# Autodesk Inventor assembly: House_Assembly
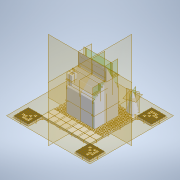
[picture p0: Inventor's stored thumbnail of the model, 180x180]
Saved by Autodesk Inventor 2022.4 (Build 264492010, 492A)
## iProperties
Created: 2025-02-20
Part Number: House_Assembly
Document SubType Name: Assembly
Designer: jan-m
Author: jan-m
## Documents named in this file (21)
- C:\School\Masterproef\3D Modellen\House_Assembly.iam
- C:\School\Masterproef\3D Modellen\Tile.ipt
- C:\School\Masterproef\3D Modellen\Tile_Connector.ipt
- C:\School\Masterproef\3D Modellen\Wall.ipt
- C:\School\Masterproef\3D Modellen\Roof_Wall_Small_Left.ipt
- C:\School\Masterproef\3D Modellen\Roof_Wall_Small_Right.ipt
- C:\School\Masterproef\3D Modellen\Roof_Wall_Large_Left.ipt
- C:\School\Masterproef\3D Modellen\Roof_Wall_Large_Right.ipt
- C:\School\Masterproef\3D Modellen\Roof_Small.ipt
- C:\School\Masterproef\3D Modellen\Roof_Large.ipt
- C:\School\Masterproef\3D Modellen\Hanging_Wall.ipt
- C:\School\Masterproef\3D Modellen\1x1_Piece.ipt
- C:\School\Masterproef\3D Modellen\Marker_Tile.ipt
- C:\School\Masterproef\3D Modellen\Tile_Cover.ipt
- C:\School\Masterproef\3D Modellen\Tree_Leaves.ipt
- C:\School\Masterproef\3D Modellen\Tree_Trunk.ipt
- C:\School\Masterproef\3D Modellen\Chimney.ipt
- C:\School\Masterproef\3D Modellen\Pin.ipt
- C:\School\Masterproef\3D Modellen\Rail_Clip_Left.ipt
- C:\School\Masterproef\3D Modellen\Rail_Clip_Right.ipt
- C:\School\Masterproef\3D Modellen\Roof_Pin_Clip.ipt
## Components (403 placed, 20 different names)
1. Wall:1 — Mate:10, Mate:11, Mate:12, Mate:40, Mate:46, Mate:59
2. Wall:2 — Mate:13, Mate:14, Mate:15, Mate:27, Mate:28, Mate:30, Mate:31, Mate:60, Mate:64, Mate:72
3. Wall:3 — Mate:19, Mate:20, Mate:21, Mate:37, Mate:42, Mate:58
4. Wall:4 — Mate:16, Mate:17, Mate:18, Mate:23, Mate:25, Mate:33, Mate:34, Mate:63, Mate:65
5. Roof_Wall_Small_Left:2 — Mate:23, Mate:25, Mate:65, Mate:80, Mate:81, Flush:6, Mate:102, Flush:12, Angle:1
6. Roof_Wall_Small_Right:2 — Mate:27, Mate:28, Mate:64, Mate:72, Mate:101, Mate:103, Flush:13, Angle:2
7. Roof_Wall_Large_Left:1 — Mate:30, Mate:31, Mate:60, Mate:106, Flush:16, Angle:5, Mate:107, Flush:17, Angle:6
8. Roof_Wall_Large_Right:1 — Mate:33, Mate:34, Mate:63, Mate:98, Mate:104, Flush:14, Angle:3, Mate:105, Flush:15, Angle:4
9. Roof_Small:1 — Mate:37, Mate:42, Mate:58, Mate:96, Mate:97, Mate:99, Mate:100
10. Roof_Large:1 — Mate:40, Mate:43, Mate:44, Mate:46, Mate:59, Flush:7
11. Hanging_Wall:1 — Mate:43, Mate:44, Flush:7
12. Tree_Leaves:1 — Mate:73, Mate:74
13. Tree_Trunk:1 — Mate:73, Mate:74, Mate:75, Mate:76, Mate:77
14. Chimney:1 — Mate:78, Mate:79, Mate:81, Flush:6
15. Pin:1 — Mate:78, Mate:79, Mate:80
16. Rail_Clip_Left:1 — Mate:96, Mate:97, Mate:98
17. Rail_Clip_Right:1 — Mate:99, Mate:100, Mate:101
18. Roof_Pin_Clip:1 — Mate:105, Flush:15, Angle:4
19. Roof_Pin_Clip:2 — Mate:106, Flush:16, Angle:5
20. Roof_Pin_Clip:3 — Mate:104, Flush:14, Angle:3
21. Roof_Pin_Clip:4 — Mate:102, Flush:12, Angle:1
22. Roof_Pin_Clip:5 — Mate:107, Flush:17, Angle:6
23. Roof_Pin_Clip:6 — Mate:103, Flush:13, Angle:2
24. Tile_Connector:2 — Mate:6, Mate:7
25. Tile:1 — Mate:2, Mate:5, Mate:6, Mate:7, Mate:16, Mate:91, Mate:92
26. Tile_Connector:1 — Mate:2, Mate:5
27. Tile_Connector:3
28. Tile:2 — Mate:10, Mate:12
29. Tile_Connector:4
30. Tile_Connector:5
31. Tile:3 — Mate:11
32. Tile_Connector:6
33. Tile_Connector:7
34. Tile:4 — Mate:13, Mate:75, Mate:76, Mate:77, Mate:94, Mate:95, Flush:11
35. Tile_Connector:8
36. Tile_Connector:9
37. Tile:5
38. Tile_Connector:10
39. Tile_Connector:11
40. Tile:6
41. Tile_Connector:12
42. Tile_Connector:13
43. Tile:7 — Mate:82, Flush:9
44. Tile_Connector:14
45. Tile_Connector:15
46. Tile:8 — Mate:15
47. Tile_Connector:16
48. Tile_Connector:17
49. Tile:9 — Mate:17, Mate:18, Mate:83, Mate:84, Flush:10, Mate:85, Mate:86
50. Tile_Connector:18
51. Tile_Connector:19
52. Tile:10 — Mate:19, Mate:21
53. Tile_Connector:20
54. Tile_Connector:21
55. Tile:11 — Mate:20
56. Tile_Connector:22
57. Tile_Connector:23
58. Tile:12 — Mate:14, Mate:88, Mate:89
59. Tile_Connector:24
60. Tile_Connector:25
61. Tile:13 — Mate:57, Mate:61, Mate:62
62. Tile_Connector:26
63. Tile_Connector:27
64. Tile:14
65. Tile_Connector:28
66. Tile_Connector:29
67. Tile:15
68. Tile_Connector:30
69. Tile_Connector:31
70. Tile:16 — Mate:66, Mate:68, Mate:70
71. Tile_Connector:32
72. Marker_Tile:1 — Mate:53, Mate:54, Flush:5, Mate:67, Mate:69, Mate:71
73. Tile_Connector:33 — Mate:66, Mate:67, Mate:68, Mate:69, Mate:70, Mate:71
74. Marker_Tile:2
75. Tile_Connector:34
76. Marker_Tile:3
77. Tile_Connector:35
78. Marker_Tile:4
79. Tile_Connector:36
80. Tile_Cover:1 — Mate:57, Mate:61, Mate:62
81. Tile_Cover:2
82. Tile_Cover:3
83. Tile_Cover:4
84. 1x1_Piece:147 — Mate:83, Mate:84, Flush:10
85. 1x1_Piece:155
86. 1x1_Piece:156
87. 1x1_Piece:157 — Mate:87
88. 1x1_Piece:158
89. 1x1_Piece:159
90. 1x1_Piece:160
91. 1x1_Piece:161
92. 1x1_Piece:162
93. 1x1_Piece:163
94. 1x1_Piece:164
95. 1x1_Piece:165
96. 1x1_Piece:166
97. 1x1_Piece:167
98. 1x1_Piece:168
99. 1x1_Piece:169
100. 1x1_Piece:170
101. 1x1_Piece:171
102. 1x1_Piece:172
103. 1x1_Piece:173
104. 1x1_Piece:174
105. 1x1_Piece:175
106. 1x1_Piece:176
107. 1x1_Piece:177
108. 1x1_Piece:178
109. 1x1_Piece:179
110. 1x1_Piece:180
111. 1x1_Piece:181
112. 1x1_Piece:182
113. 1x1_Piece:183
114. 1x1_Piece:184
115. 1x1_Piece:185
116. 1x1_Piece:186
117. 1x1_Piece:187
118. 1x1_Piece:188
119. 1x1_Piece:189
120. 1x1_Piece:190
121. 1x1_Piece:191
122. 1x1_Piece:192
123. 1x1_Piece:193
124. 1x1_Piece:194
125. 1x1_Piece:195
126. 1x1_Piece:196
127. 1x1_Piece:197
128. 1x1_Piece:198
129. 1x1_Piece:199
130. 1x1_Piece:200
131. 1x1_Piece:201 — Mate:93
132. 1x1_Piece:202
133. 1x1_Piece:203
134. 1x1_Piece:204
135. 1x1_Piece:205
136. 1x1_Piece:206
137. 1x1_Piece:207
138. 1x1_Piece:208
139. 1x1_Piece:209
140. 1x1_Piece:210
141. 1x1_Piece:211
142. 1x1_Piece:212
143. 1x1_Piece:213
144. 1x1_Piece:146 — Mate:85, Mate:86, Mate:87
145. 1x1_Piece:214
146. 1x1_Piece:215
147. 1x1_Piece:216
148. 1x1_Piece:217
149. 1x1_Piece:218
150. 1x1_Piece:219
151. 1x1_Piece:220
152. 1x1_Piece:221
153. 1x1_Piece:222
154. 1x1_Piece:223
155. 1x1_Piece:224 — Mate:90
156. 1x1_Piece:151 — Mate:88, Mate:89, Mate:90
157. 1x1_Piece:225
158. 1x1_Piece:226
159. 1x1_Piece:227
160. 1x1_Piece:228
161. 1x1_Piece:229
162. 1x1_Piece:230
163. 1x1_Piece:231
164. 1x1_Piece:232
165. 1x1_Piece:233
166. 1x1_Piece:234
167. 1x1_Piece:235
168. 1x1_Piece:236
169. 1x1_Piece:237
170. 1x1_Piece:238
171. 1x1_Piece:239
172. 1x1_Piece:240
173. 1x1_Piece:241
174. 1x1_Piece:242
175. 1x1_Piece:243
176. 1x1_Piece:244
177. 1x1_Piece:245
178. 1x1_Piece:246
179. 1x1_Piece:247
180. 1x1_Piece:248
181. 1x1_Piece:249
182. 1x1_Piece:250
183. 1x1_Piece:251
184. 1x1_Piece:252
185. 1x1_Piece:253
186. 1x1_Piece:254
187. 1x1_Piece:255
188. 1x1_Piece:256
189. 1x1_Piece:257
190. 1x1_Piece:258
191. 1x1_Piece:259
192. 1x1_Piece:260
193. 1x1_Piece:261
194. 1x1_Piece:262
195. 1x1_Piece:263
196. 1x1_Piece:264
197. 1x1_Piece:265
198. 1x1_Piece:266
199. 1x1_Piece:267
200. 1x1_Piece:268
201. 1x1_Piece:269
202. 1x1_Piece:270
203. 1x1_Piece:271
204. 1x1_Piece:272
205. 1x1_Piece:273
206. 1x1_Piece:274
207. 1x1_Piece:275
208. 1x1_Piece:145 — Mate:91, Mate:92, Mate:93
209. 1x1_Piece:276
210. 1x1_Piece:277
211. 1x1_Piece:278
212. 1x1_Piece:279
213. 1x1_Piece:280
214. 1x1_Piece:281
215. 1x1_Piece:282
216. 1x1_Piece:283
217. 1x1_Piece:284
218. 1x1_Piece:285
219. 1x1_Piece:286
220. 1x1_Piece:287
221. 1x1_Piece:288
222. 1x1_Piece:289
223. 1x1_Piece:290
224. 1x1_Piece:291
225. 1x1_Piece:292
226. 1x1_Piece:293
227. 1x1_Piece:294
228. 1x1_Piece:295
229. 1x1_Piece:296
230. 1x1_Piece:297
231. 1x1_Piece:298
232. 1x1_Piece:299
233. 1x1_Piece:300
234. 1x1_Piece:301
235. 1x1_Piece:302
236. 1x1_Piece:303
237. 1x1_Piece:304
238. 1x1_Piece:305
239. 1x1_Piece:306
240. 1x1_Piece:307
241. 1x1_Piece:308
242. 1x1_Piece:309
243. 1x1_Piece:310
244. 1x1_Piece:311
245. 1x1_Piece:312
246. 1x1_Piece:313
247. 1x1_Piece:314
248. 1x1_Piece:315
249. 1x1_Piece:316
250. 1x1_Piece:317
251. 1x1_Piece:318
252. 1x1_Piece:319
253. 1x1_Piece:320
254. 1x1_Piece:321
255. 1x1_Piece:322
256. 1x1_Piece:148 — Mate:94, Mate:95, Flush:11
257. 1x1_Piece:323
258. 1x1_Piece:324
259. 1x1_Piece:325
260. 1x1_Piece:1 — Mate:53, Mate:54, Flush:5, Flush:8
261. 1x1_Piece:2
262. 1x1_Piece:3
263. 1x1_Piece:4
264. 1x1_Piece:5
265. 1x1_Piece:6
266. 1x1_Piece:7
267. 1x1_Piece:8
268. 1x1_Piece:9
269. 1x1_Piece:10
270. 1x1_Piece:11
271. 1x1_Piece:12
272. 1x1_Piece:13
273. 1x1_Piece:14
274. 1x1_Piece:15
275. 1x1_Piece:16
276. 1x1_Piece:17
277. 1x1_Piece:18
278. 1x1_Piece:19
279. 1x1_Piece:20
280. 1x1_Piece:21
281. 1x1_Piece:22
282. 1x1_Piece:23
283. 1x1_Piece:24
284. 1x1_Piece:25
285. 1x1_Piece:26
286. 1x1_Piece:27
287. 1x1_Piece:28
288. 1x1_Piece:29
289. 1x1_Piece:30
290. 1x1_Piece:31
291. 1x1_Piece:32
292. 1x1_Piece:33
293. 1x1_Piece:34
294. 1x1_Piece:35
295. 1x1_Piece:36
296. 1x1_Piece:37
297. 1x1_Piece:38
298. 1x1_Piece:39
299. 1x1_Piece:40
300. 1x1_Piece:41
301. 1x1_Piece:42
302. 1x1_Piece:43
303. 1x1_Piece:44
304. 1x1_Piece:45
305. 1x1_Piece:46
306. 1x1_Piece:47
307. 1x1_Piece:48
308. 1x1_Piece:49
309. 1x1_Piece:50
310. 1x1_Piece:51
311. 1x1_Piece:52
312. 1x1_Piece:53
313. 1x1_Piece:54
314. 1x1_Piece:55
315. 1x1_Piece:56
316. 1x1_Piece:57
317. 1x1_Piece:58
318. 1x1_Piece:59
319. 1x1_Piece:60
320. 1x1_Piece:61
321. 1x1_Piece:62
322. 1x1_Piece:63
323. 1x1_Piece:64
324. 1x1_Piece:65
325. 1x1_Piece:66
326. 1x1_Piece:67
327. 1x1_Piece:68
328. 1x1_Piece:69
329. 1x1_Piece:70
330. 1x1_Piece:71
331. 1x1_Piece:72
332. 1x1_Piece:73
333. 1x1_Piece:74
334. 1x1_Piece:75
335. 1x1_Piece:76
336. 1x1_Piece:77
337. 1x1_Piece:78
338. 1x1_Piece:79
339. 1x1_Piece:80
340. 1x1_Piece:81
341. 1x1_Piece:82
342. 1x1_Piece:83
343. 1x1_Piece:84
344. 1x1_Piece:85
345. 1x1_Piece:86
346. 1x1_Piece:87
347. 1x1_Piece:88
348. 1x1_Piece:89
349. 1x1_Piece:90
350. 1x1_Piece:91
351. 1x1_Piece:92
352. 1x1_Piece:93
353. 1x1_Piece:94
354. 1x1_Piece:95
355. 1x1_Piece:96
356. 1x1_Piece:97
357. 1x1_Piece:98
358. 1x1_Piece:99
359. 1x1_Piece:100
360. 1x1_Piece:101
361. 1x1_Piece:102
362. 1x1_Piece:103
363. 1x1_Piece:104
364. 1x1_Piece:105
365. 1x1_Piece:106
366. 1x1_Piece:107
367. 1x1_Piece:108
368. 1x1_Piece:109
369. 1x1_Piece:110
370. 1x1_Piece:111
371. 1x1_Piece:112
372. 1x1_Piece:113
373. 1x1_Piece:114
374. 1x1_Piece:115
375. 1x1_Piece:116
376. 1x1_Piece:117
377. 1x1_Piece:118
378. 1x1_Piece:119
379. 1x1_Piece:120
380. 1x1_Piece:121
381. 1x1_Piece:122
382. 1x1_Piece:123
383. 1x1_Piece:124
384. 1x1_Piece:125
385. 1x1_Piece:126
386. 1x1_Piece:127
387. 1x1_Piece:128
388. 1x1_Piece:129
389. 1x1_Piece:130
390. 1x1_Piece:131
391. 1x1_Piece:132
392. 1x1_Piece:133
393. 1x1_Piece:134
394. 1x1_Piece:135
395. 1x1_Piece:136
396. 1x1_Piece:137
397. 1x1_Piece:138
398. 1x1_Piece:139
399. 1x1_Piece:140
400. 1x1_Piece:141
401. 1x1_Piece:142
402. 1x1_Piece:143
403. 1x1_Piece:144
## Component patterns: (16 elements, first: Tile_Connector:2 + Tile:1 + Tile_Connector:1), (4 elements, first: Marker_Tile:1 + Tile_Connector:33), (4 elements, first: Tile_Cover:1), (60 elements, first: 1x1_Piece:147), (12 elements, first: 1x1_Piece:146), (52 elements, first: 1x1_Piece:151), (48 elements, first: 1x1_Piece:145), (4 elements, first: 1x1_Piece:148), (36 elements, first: 1x1_Piece:1), Component Pattern 2:2 (36 elements), Component Pattern 2:3 (36 elements), Component Pattern 2:4 (36 elements)
## Relationships (102: Mate 83, Flush 13, Angle 6)
- Mate:2: Tile:1 ↔ Tile_Connector:1
- Mate:5: Tile:1 ↔ Tile_Connector:1
- Mate:6: Tile_Connector:2 ↔ Tile:1
- Mate:7: Tile_Connector:2 ↔ Tile:1
- Mate:10: Wall:1 ↔ Tile:2
- Mate:11: Wall:1 ↔ Tile:3
- Mate:12: Wall:1 ↔ Tile:2
- Mate:13: Wall:2 ↔ Tile:4
- Mate:14: Wall:2 ↔ Tile:12
- Mate:15: Wall:2 ↔ Tile:8
- Mate:16: Wall:4 ↔ Tile:1
- Mate:17: Wall:4 ↔ Tile:9
- Mate:18: Wall:4 ↔ Tile:9
- Mate:19: Wall:3 ↔ Tile:10
- Mate:20: Wall:3 ↔ Tile:11
- Mate:21: Wall:3 ↔ Tile:10
- Mate:23: Wall:4 ↔ Roof_Wall_Small_Left:2
- Mate:25: Wall:4 ↔ Roof_Wall_Small_Left:2
- Mate:27: Wall:2 ↔ Roof_Wall_Small_Right:2
- Mate:28: Wall:2 ↔ Roof_Wall_Small_Right:2
- Mate:30: Wall:2 ↔ Roof_Wall_Large_Left:1
- Mate:31: Wall:2 ↔ Roof_Wall_Large_Left:1
- Mate:33: Wall:4 ↔ Roof_Wall_Large_Right:1
- Mate:34: Wall:4 ↔ Roof_Wall_Large_Right:1
- Mate:37: Wall:3 ↔ Roof_Small:1
- Mate:40: Wall:1 ↔ Roof_Large:1
- Mate:42: Wall:3 ↔ Roof_Small:1
- Mate:43: Roof_Large:1 ↔ Hanging_Wall:1
- Mate:44: Roof_Large:1 ↔ Hanging_Wall:1
- Mate:46: Wall:1 ↔ Roof_Large:1
- Mate:53: Marker_Tile:1 ↔ 1x1_Piece:1
- Mate:54: Marker_Tile:1 ↔ 1x1_Piece:1
- Mate:57: Tile:13 ↔ Tile_Cover:1
- Mate:58: Wall:3 ↔ Roof_Small:1
- Mate:59: Wall:1 ↔ Roof_Large:1
- Flush:5: Marker_Tile:1 ↔ 1x1_Piece:1
- Mate:60: Wall:2 ↔ Roof_Wall_Large_Left:1
- Mate:61: Tile:13 ↔ Tile_Cover:1
- Mate:62: Tile:13 ↔ Tile_Cover:1
- Mate:63: Wall:4 ↔ Roof_Wall_Large_Right:1
- Mate:64: Wall:2 ↔ Roof_Wall_Small_Right:2
- Mate:65: Wall:4 ↔ Roof_Wall_Small_Left:2
- Mate:66: Tile:16 ↔ Tile_Connector:33
- Mate:67: Marker_Tile:1 ↔ Tile_Connector:33
- Mate:68: Tile:16 ↔ Tile_Connector:33
- Mate:69: Marker_Tile:1 ↔ Tile_Connector:33
- Mate:70: Tile:16 ↔ Tile_Connector:33
- Mate:71: Marker_Tile:1 ↔ Tile_Connector:33
- Mate:72: Wall:2 ↔ Roof_Wall_Small_Right:2
- Mate:73: Tree_Leaves:1 ↔ Tree_Trunk:1
- Mate:74: Tree_Leaves:1 ↔ Tree_Trunk:1
- Mate:75: Tree_Trunk:1 ↔ Tile:4
- Mate:76: Tree_Trunk:1 ↔ Tile:4
- Mate:77: Tree_Trunk:1 ↔ Tile:4
- Mate:78: Chimney:1 ↔ Pin:1
- Mate:79: Chimney:1 ↔ Pin:1
- Mate:80: Roof_Wall_Small_Left:2 ↔ Pin:1
- Mate:81: Roof_Wall_Small_Left:2 ↔ Chimney:1
- Flush:6: Roof_Wall_Small_Left:2 ↔ Chimney:1
- Flush:7: Roof_Large:1 ↔ Hanging_Wall:1
- Mate:82: Tile:7
- Flush:8: 1x1_Piece:1
- Flush:9: Tile:7
- Mate:83: Tile:9 ↔ 1x1_Piece:147
- Mate:84: Tile:9 ↔ 1x1_Piece:147
- Flush:10: Tile:9 ↔ 1x1_Piece:147
- Mate:85: Tile:9 ↔ 1x1_Piece:146
- Mate:86: Tile:9 ↔ 1x1_Piece:146
- Mate:87: 1x1_Piece:157 ↔ 1x1_Piece:146
- Mate:88: Tile:12 ↔ 1x1_Piece:151
- Mate:89: Tile:12 ↔ 1x1_Piece:151
- Mate:90: 1x1_Piece:224 ↔ 1x1_Piece:151
- Mate:91: Tile:1 ↔ 1x1_Piece:145
- Mate:92: Tile:1 ↔ 1x1_Piece:145
- Mate:93: 1x1_Piece:201 ↔ 1x1_Piece:145
- Mate:94: Tile:4 ↔ 1x1_Piece:148
- Mate:95: Tile:4 ↔ 1x1_Piece:148
- Flush:11: Tile:4 ↔ 1x1_Piece:148
- Mate:96: Roof_Small:1 ↔ Rail_Clip_Left:1
- Mate:97: Roof_Small:1 ↔ Rail_Clip_Left:1
- Mate:98: Roof_Wall_Large_Right:1 ↔ Rail_Clip_Left:1
- Mate:99: Roof_Small:1 ↔ Rail_Clip_Right:1
- Mate:100: Roof_Small:1 ↔ Rail_Clip_Right:1
- Mate:101: Roof_Wall_Small_Right:2 ↔ Rail_Clip_Right:1
- Mate:102: Roof_Wall_Small_Left:2 ↔ Roof_Pin_Clip:4
- Flush:12: Roof_Wall_Small_Left:2 ↔ Roof_Pin_Clip:4
- Mate:103: Roof_Wall_Small_Right:2 ↔ Roof_Pin_Clip:6
- Flush:13: Roof_Wall_Small_Right:2 ↔ Roof_Pin_Clip:6
- Angle:1 (90 deg): Roof_Wall_Small_Left:2 ↔ Roof_Pin_Clip:4
- Angle:2 (90 deg): Roof_Wall_Small_Right:2 ↔ Roof_Pin_Clip:6
- Mate:104: Roof_Wall_Large_Right:1 ↔ Roof_Pin_Clip:3
- Flush:14: Roof_Wall_Large_Right:1 ↔ Roof_Pin_Clip:3
- Angle:3 (90 deg): Roof_Wall_Large_Right:1 ↔ Roof_Pin_Clip:3
- Mate:105: Roof_Wall_Large_Right:1 ↔ Roof_Pin_Clip:1
- Flush:15: Roof_Wall_Large_Right:1 ↔ Roof_Pin_Clip:1
- Angle:4 (90 deg): Roof_Wall_Large_Right:1 ↔ Roof_Pin_Clip:1
- Mate:106: Roof_Wall_Large_Left:1 ↔ Roof_Pin_Clip:2
- Flush:16: Roof_Wall_Large_Left:1 ↔ Roof_Pin_Clip:2
- Angle:5 (270 deg): Roof_Wall_Large_Left:1 ↔ Roof_Pin_Clip:2
- Mate:107: Roof_Wall_Large_Left:1 ↔ Roof_Pin_Clip:5
- Flush:17: Roof_Wall_Large_Left:1 ↔ Roof_Pin_Clip:5
- Angle:6 (90 deg): Roof_Wall_Large_Left:1 ↔ Roof_Pin_Clip:5
